# Autodesk Inventor assembly: ass_1
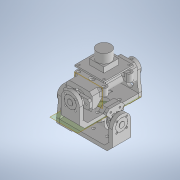
[picture p0: Inventor's stored thumbnail of the model, 180x180]
Saved by Autodesk Inventor 2020 (Build 240168000, 168)
## iProperties
Created: 2020-05-02
Part Number: ass_1
Document SubType Name: Assembly
Designer: psrobotics
Author: psrobotics
## Documents named in this file (12)
- F:\projects-3\pan_tilt\hardware\ass_1.iam
- F:\projects-3\pan_tilt\hardware\maxon_motor.ipt
- F:\projects-3\pan_tilt\hardware\holder_1.ipt
- F:\projects-3\pan_tilt\hardware\cam_1.ipt
- F:\projects-3\pan_tilt\hardware\pin_1.ipt
- F:\projects-3\pan_tilt\hardware\bearing_6_13_3.5.ipt
- F:\projects-3\pan_tilt\hardware\ma.ipt
- F:\projects-3\pan_tilt\hardware\holder_2.ipt
- F:\projects-3\pan_tilt\hardware\holder_3.ipt
- F:\projects-3\pan_tilt\hardware\pin_2.ipt
- F:\projects-3\pan_tilt\hardware\mpin_holder_1.ipt
- F:\projects-3\pan_tilt\hardware\holder_4.ipt
## Components (17 placed, 11 different names)
1. maxon_motor:1 — Flush:1, Insert:1, Insert:2
2. holder_1:1 — Flush:1, Insert:1, Insert:2, Mate:1, Flush:2, Flush:3, Insert:3, Insert:4, Angle:1
3. cam_1:1 — Mate:1, Flush:2, Flush:3
4. pin_1:1 — Insert:3, Insert:4, Insert:5, Insert:7
5. bearing_6_13_3.5:1 — Insert:5, Insert:6
6. bearing_6_13_3.5:2 — Insert:6, Flush:4, Insert:16
7. ma:1 — Insert:7
8. holder_2:1 — Flush:4, Flush:5, Tangent:1, Tangent:2, Flush:6, Angle:1, Insert:8, Flush:7, Insert:9, Insert:10, Flush:8, Insert:11, Insert:12, Insert:16, Angle:2
9. maxon_motor:2 — Flush:5, Tangent:1, Tangent:2
10. holder_3:1 — Flush:6, Insert:8
11. pin_2:1 — Flush:7, Insert:9, Insert:10, Insert:13, Insert:17
12. mpin_holder_1:1 — Flush:8, Insert:11, Insert:12
13. holder_4:1 — Insert:15, Flush:9, Mate:2, Flush:10, Angle:2
14. bearing_6_13_3.5:3 — Insert:14, Insert:15
15. bearing_6_13_3.5:4 — Insert:13, Insert:14
16. mpin_holder_1:2 — Flush:9, Mate:2, Flush:10
17. ma:2 — Insert:17
## Relationships (33: Insert 17, Flush 10, Mate 2, Tangent 2, Angle 2)
- Flush:1: maxon_motor:1 ↔ holder_1:1
- Insert:1: maxon_motor:1 ↔ holder_1:1
- Insert:2: maxon_motor:1 ↔ holder_1:1
- Mate:1 (5 mm): holder_1:1 ↔ cam_1:1
- Flush:2 (10 mm): holder_1:1 ↔ cam_1:1
- Flush:3 (-5.5 mm): holder_1:1 ↔ cam_1:1
- Insert:3: holder_1:1 ↔ pin_1:1
- Insert:4: holder_1:1 ↔ pin_1:1
- Insert:5: pin_1:1 ↔ bearing_6_13_3.5:1
- Insert:6: bearing_6_13_3.5:1 ↔ bearing_6_13_3.5:2
- Insert:7: pin_1:1 ↔ ma:1
- Flush:4: bearing_6_13_3.5:2 ↔ holder_2:1
- Flush:5: holder_2:1 ↔ maxon_motor:2
- Tangent:1: holder_2:1 ↔ maxon_motor:2
- Tangent:2 (-43 mm): holder_2:1 ↔ maxon_motor:2
- Flush:6: holder_2:1 ↔ holder_3:1
- Angle:1 (0 deg): holder_1:1 ↔ holder_2:1
- Insert:8: holder_2:1 ↔ holder_3:1
- Flush:7: holder_2:1 ↔ pin_2:1
- Insert:9: holder_2:1 ↔ pin_2:1
- Insert:10: holder_2:1 ↔ pin_2:1
- Flush:8: holder_2:1 ↔ mpin_holder_1:1
- Insert:11: holder_2:1 ↔ mpin_holder_1:1
- Insert:12: holder_2:1 ↔ mpin_holder_1:1
- Insert:13: pin_2:1 ↔ bearing_6_13_3.5:4
- Insert:14: bearing_6_13_3.5:3 ↔ bearing_6_13_3.5:4
- Insert:15: holder_4:1 ↔ bearing_6_13_3.5:3
- Insert:16: bearing_6_13_3.5:2 ↔ holder_2:1
- Flush:9: holder_4:1 ↔ mpin_holder_1:2
- Mate:2: holder_4:1 ↔ mpin_holder_1:2
- Flush:10: holder_4:1 ↔ mpin_holder_1:2
- Insert:17: pin_2:1 ↔ ma:2
- Angle:2 (0 deg): holder_2:1 ↔ holder_4:1
